# Autodesk Inventor assembly: KB33-046-004 - Внешний корпус
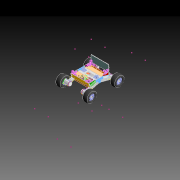
[picture p0: Inventor's stored thumbnail of the model, 180x180]
Saved by Autodesk Inventor 2020 (Build 240168000, 168)
## iProperties
Created: 2021-06-25
Part Number: KB33-046-004 - Внешний корпус
Document SubType Name: Assembly
Designer: Петров Иван
Mass: 3036.48 g
Surface Area: 14093.4 cm^2
Volume: 2856.02 cm^3
Density: 1.06319 g/cm^3
Author: Петров Иван
## Documents named in this file (32)
- E:\IVAN\Ivan_desktop\Kvantorium\Projects\RoboPatrol\design\KB33-046-004 - Внешний корпус.iam
- E:\IVAN\Ivan_desktop\Kvantorium\Projects\RoboPatrol\design\KB33-046-004-001 - Центральная пластина.ipt
- E:\IVAN\Ivan_desktop\Kvantorium\Projects\RoboPatrol\design\KB33-046-004-002 - Передняя пластина.ipt
- E:\IVAN\Ivan_desktop\Kvantorium\Projects\RoboPatrol\design\KB33-046-001 - Ходовая часть.iam
- E:\IVAN\Ivan_desktop\Kvantorium\Projects\RoboPatrol\design\KB33-046-004-003 - Задняя пластина.ipt
- E:\IVAN\Ivan_desktop\Kvantorium\Projects\RoboPatrol\design\KB33-046-004-004 - Центральная верхняя пластина.ipt
- E:\IVAN\Ivan_desktop\Kvantorium\Projects\RoboPatrol\design\KB33-046-004-005 - Лицевая наклонная пластина.ipt
- E:\IVAN\Ivan_desktop\Kvantorium\Projects\RoboPatrol\design\KB33-046-004-006 - Задняя наклонная пластина.ipt
- E:\IVAN\Ivan_desktop\Kvantorium\Projects\RoboPatrol\design\KB33-046-004-007 - Центральная левая боковая пластина.ipt
- E:\IVAN\Ivan_desktop\Kvantorium\Projects\RoboPatrol\design\KB33-046-004-008 - Центральная правая боковая пластина.ipt
- E:\IVAN\Ivan_desktop\Kvantorium\Projects\RoboPatrol\design\KB33-046-004-009 - Передняя левая боковая пластина.ipt
- E:\IVAN\Ivan_desktop\Kvantorium\Projects\RoboPatrol\design\KB33-046-004-010 - Передняя правая боковая пластина.ipt
- E:\IVAN\Ivan_desktop\Kvantorium\Projects\RoboPatrol\design\KB33-046-004-011 - Задняя правая боковая пластина.ipt
- E:\IVAN\Ivan_desktop\Kvantorium\Projects\RoboPatrol\design\KB33-046-004-012 - Задняя левая боковая пластина.ipt
- E:\IVAN\Ivan_desktop\Kvantorium\Projects\RoboPatrol\design\KB33-046-004-013 - Уголок.ipt
- E:\IVAN\Ivan_desktop\Kvantorium\Projects\RoboPatrol\design\KB33-046-004-013 - Уголок зеркальный.ipt
- E:\IVAN\Ivan_desktop\Kvantorium\Projects\RoboPatrol\design\standart_components\JetsonNano\Jetson nano_fixed.iam
- E:\IVAN\Ivan_desktop\Kvantorium\Projects\RoboPatrol\design\KB33-046-004-014 - Лицевая вертикальня пластина.ipt
- E:\IVAN\Ivan_desktop\Kvantorium\Projects\RoboPatrol\design\KB33-046-004-015 - Задняя вертикальня пластина.ipt
- E:\IVAN\Ivan_desktop\Kvantorium\Projects\RoboPatrol\design\KB33-046-004-016 - Крышка.ipt
- E:\IVAN\Ivan_desktop\Kvantorium\Projects\RoboPatrol\design\KB33-046-004-017 - Крышка наклонная.ipt
- E:\IVAN\Ivan_desktop\Kvantorium\Projects\RoboPatrol\design\KB33-046-004-018 - Полка электроники.ipt
- E:\IVAN\Ivan_desktop\Kvantorium\Projects\RoboPatrol\design\standart_components\Lidar\RPLIDAR A2.iam
- E:\IVAN\Ivan_desktop\Kvantorium\Projects\RoboPatrol\design\standart_components\L298N\L298N_V2.ipt
- E:\IVAN\Ivan_desktop\Kvantorium\Projects\RoboPatrol\design\KB33-046-004-019 - Площадка под драйверы.ipt
- E:\IVAN\Ivan_desktop\Kvantorium\Projects\RoboPatrol\design\KB33-046-005 - Контроллер СНУ.iam
- E:\IVAN\Ivan_desktop\Kvantorium\Projects\RoboPatrol\design\KB33-046-007 - Контроллер АКБ.iam
- E:\IVAN\Ivan_desktop\Kvantorium\Projects\RoboPatrol\design\standart_components\Realsense\D400\IntelRealsense_D435_Multibody.ipt
- E:\IVAN\Ivan_desktop\Kvantorium\Projects\RoboPatrol\design\KB33-046-004-020 - Крепление глубинной камеры.ipt
- E:\IVAN\Ivan_desktop\Kvantorium\Projects\RoboPatrol\design\standart_components\TP_LINK_MR3023.ipt
- E:\IVAN\Ivan_desktop\Kvantorium\Projects\RoboPatrol\design\KB33-046-009 - Колпак лидара.iam
- E:\IVAN\Ivan_desktop\Kvantorium\Projects\RoboPatrol\design\KB33-046-008 - Блок АКБ.iam
## Components (35 placed, 31 different names)
1. KB33-046-004-001 - Центральная пластина:1 — Совмещение:1, Совмещение:2, Совмещение:3
2. KB33-046-004-002 - Передняя пластина:1 — Совмещение:4, Совмещение:5, Совмещение:6, Совмещение:80, Совмещение:100
3. KB33-046-001 - Ходовая часть:1 [sub-assembly] — Совмещение:1, Совмещение:2, Совмещение:3, Совмещение:4, Совмещение:5, Совмещение:6, Совмещение:7, Совмещение:8, Совмещение:9, Совмещение:10, Совмещение:11, Совмещение:12, Заподлицо:1, Совмещение:13, Совмещение:15, Совмещение:16, Совмещение:18, Совмещение:19, Совмещение:20, Совмещение:21, Совмещение:22, Совмещение:23, Заподлицо:2, Совмещение:24, Совмещение:25, Совмещение:26, Совмещение:27, Совмещение:28, Совмещение:29, Совмещение:30, Совмещение:31, Совмещение:32, Совмещение:33, Совмещение:34, Касательность:2, Совмещение:61, Совмещение:62, Совмещение:72, Заподлицо:16, Совмещение:101, Совмещение:102, Совмещение:104, Совмещение:105
4. KB33-046-004-003 - Задняя пластина:1 — Совмещение:7, Совмещение:8, Совмещение:9, Совмещение:103
5. KB33-046-004-004 - Центральная верхняя пластина:1 — Совмещение:10, Совмещение:11, Совмещение:12, Совмещение:73
6. KB33-046-004-005 - Лицевая наклонная пластина:1 — Заподлицо:1, Совмещение:13, Совмещение:36, Совмещение:40, Совмещение:62, Совмещение:81
7. KB33-046-004-006 - Задняя наклонная пластина:1 — Совмещение:15, Совмещение:16, Совмещение:38, Совмещение:42, Совмещение:61
8. KB33-046-004-007 - Центральная левая боковая пластина:1 — Совмещение:18, Совмещение:19, Совмещение:20
9. KB33-046-004-008 - Центральная правая боковая пластина:1 — Совмещение:21, Совмещение:22, Совмещение:23, Заподлицо:11, Заподлицо:12, Заподлицо:14, Совмещение:54
10. KB33-046-004-009 - Передняя левая боковая пластина:1 — Заподлицо:2, Совмещение:33, Совмещение:34, Совмещение:35, Заподлицо:3
11. KB33-046-004-010 - Передняя правая боковая пластина:1 — Совмещение:24, Совмещение:25, Совмещение:26, Совмещение:39, Заподлицо:5
12. KB33-046-004-011 - Задняя правая боковая пластина:1 — Совмещение:27, Совмещение:28, Совмещение:29, Совмещение:37, Заподлицо:4
13. KB33-046-004-012 - Задняя левая боковая пластина:1 — Совмещение:30, Совмещение:31, Совмещение:32, Совмещение:41, Заподлицо:6
14. KB33-046-004-013 - Уголок:1 — Совмещение:35, Совмещение:36, Заподлицо:3, Угол:2
15. KB33-046-004-013 - Уголок:2 — Совмещение:37, Совмещение:38, Заподлицо:4, Совмещение:49, Совмещение:50, Заподлицо:15, Угол:4
16. KB33-046-004-013 - Уголок зеркальный:1 — Совмещение:39, Заподлицо:5, Совмещение:40, Заподлицо:8, Заподлицо:9, Совмещение:48, Совмещение:63, Совмещение:82
17. KB33-046-004-013 - Уголок зеркальный:2 — Совмещение:41, Заподлицо:6, Совмещение:42, Угол:1, Совмещение:64
18. Jetson nano_fixed:1 [sub-assembly] — Совмещение:55, Совмещение:92, Совмещение:93, Совмещение:95
19. KB33-046-004-014 - Лицевая вертикальня пластина:1 — Заподлицо:8, Заподлицо:9, Совмещение:48
20. KB33-046-004-015 - Задняя вертикальня пластина:1 — Совмещение:49, Совмещение:50, Заподлицо:10, Заподлицо:13
21. KB33-046-004-016 - Крышка:1 — Заподлицо:10, Заподлицо:12, Заподлицо:13, Совмещение:67, Касательность:3, Угол:3, Совмещение:98, Угол:6
22. KB33-046-004-017 - Крышка наклонная:1 — Заподлицо:11, Заподлицо:14, Совмещение:54
23. KB33-046-004-018 - Полка электроники:1 — Заподлицо:15, Совмещение:55, Совмещение:63, Совмещение:64, Совмещение:89, Совмещение:95, Заподлицо:21
24. RPLIDAR A2:1 [sub-assembly] — Совмещение:67, Касательность:3, Угол:3, Совмещение:99
25. L298N_V2:1 — Угол:4, Угол:5, Заподлицо:17, Совмещение:75, Совмещение:76, Совмещение:79
26. L298N_V2:2 — Угол:5, Заподлицо:18, Совмещение:74, Совмещение:76
27. KB33-046-004-019 - Площадка под драйверы:1 — Совмещение:72, Совмещение:73, Заподлицо:16, Заподлицо:17, Заподлицо:18, Совмещение:74, Совмещение:75, Совмещение:77, Совмещение:78
28. main_pcb.brd:1 [sub-assembly] — Совмещение:80, Совмещение:81, Совмещение:82, Совмещение:87, Заподлицо:19, Заподлицо:20
29. BATTERIES_CONTROLLER.brd:1 [sub-assembly] — Совмещение:87, Заподлицо:19, Заподлицо:20
30. IntelRealsense_D435_Multibody:1 — Совмещение:90, Совмещение:91
31. KB33-046-004-020 - Крепление глубинной камеры:1 — Совмещение:89, Совмещение:90, Совмещение:91, Совмещение:92, Совмещение:93, Заподлицо:21
32. TP_LINK_MR3023:1 — Совмещение:106, Совмещение:107, Угол:7
33. KB33-046-009 - Колпак лидара:1 [sub-assembly] — Совмещение:98, Совмещение:99, Угол:6, Совмещение:106, Совмещение:107, Угол:7
34. KB33-046-008 - Блок АКБ:1 [sub-assembly] — Совмещение:100, Совмещение:101, Совмещение:102
35. KB33-046-008 - Блок АКБ:2 [sub-assembly] — Совмещение:103, Совмещение:104, Совмещение:105
## Relationships (107: Mate 78, Flush 20, Angle 7, Tangent 2)
- Совмещение:1 [Mate]: KB33-046-004-001 - Центральная пластина:1 ↔ KB33-046-001 - Ходовая часть:1
- Совмещение:2 [Mate]: KB33-046-004-001 - Центральная пластина:1 ↔ KB33-046-001 - Ходовая часть:1
- Совмещение:3 [Mate]: KB33-046-004-001 - Центральная пластина:1 ↔ KB33-046-001 - Ходовая часть:1
- Совмещение:4 [Mate]: KB33-046-004-002 - Передняя пластина:1 ↔ KB33-046-001 - Ходовая часть:1
- Совмещение:5 [Mate]: KB33-046-004-002 - Передняя пластина:1 ↔ KB33-046-001 - Ходовая часть:1
- Совмещение:6 [Mate]: KB33-046-004-002 - Передняя пластина:1 ↔ KB33-046-001 - Ходовая часть:1
- Совмещение:7 [Mate]: KB33-046-001 - Ходовая часть:1 ↔ KB33-046-004-003 - Задняя пластина:1
- Совмещение:8 [Mate]: KB33-046-001 - Ходовая часть:1 ↔ KB33-046-004-003 - Задняя пластина:1
- Совмещение:9 [Mate]: KB33-046-001 - Ходовая часть:1 ↔ KB33-046-004-003 - Задняя пластина:1
- Совмещение:10 [Mate]: KB33-046-001 - Ходовая часть:1 ↔ KB33-046-004-004 - Центральная верхняя пластина:1
- Совмещение:11 [Mate]: KB33-046-001 - Ходовая часть:1 ↔ KB33-046-004-004 - Центральная верхняя пластина:1
- Совмещение:12 [Mate]: KB33-046-001 - Ходовая часть:1 ↔ KB33-046-004-004 - Центральная верхняя пластина:1
- Заподлицо:1 [Flush]: KB33-046-001 - Ходовая часть:1 ↔ KB33-046-004-005 - Лицевая наклонная пластина:1
- Совмещение:13 [Mate]: KB33-046-001 - Ходовая часть:1 ↔ KB33-046-004-005 - Лицевая наклонная пластина:1
- Совмещение:15 [Mate]: KB33-046-001 - Ходовая часть:1 ↔ KB33-046-004-006 - Задняя наклонная пластина:1
- Совмещение:16 [Mate]: KB33-046-001 - Ходовая часть:1 ↔ KB33-046-004-006 - Задняя наклонная пластина:1
- Совмещение:18 [Mate]: KB33-046-001 - Ходовая часть:1 ↔ KB33-046-004-007 - Центральная левая боковая пластина:1
- Совмещение:19 [Mate]: KB33-046-001 - Ходовая часть:1 ↔ KB33-046-004-007 - Центральная левая боковая пластина:1
- Совмещение:20 [Mate]: KB33-046-001 - Ходовая часть:1 ↔ KB33-046-004-007 - Центральная левая боковая пластина:1
- Совмещение:21 [Mate]: KB33-046-001 - Ходовая часть:1 ↔ KB33-046-004-008 - Центральная правая боковая пластина:1
- Совмещение:22 [Mate]: KB33-046-001 - Ходовая часть:1 ↔ KB33-046-004-008 - Центральная правая боковая пластина:1
- Совмещение:23 [Mate]: KB33-046-001 - Ходовая часть:1 ↔ KB33-046-004-008 - Центральная правая боковая пластина:1
- Заподлицо:2 [Flush]: KB33-046-001 - Ходовая часть:1 ↔ KB33-046-004-009 - Передняя левая боковая пластина:1
- Совмещение:24 [Mate]: KB33-046-001 - Ходовая часть:1 ↔ KB33-046-004-010 - Передняя правая боковая пластина:1
- Совмещение:25 [Mate]: KB33-046-001 - Ходовая часть:1 ↔ KB33-046-004-010 - Передняя правая боковая пластина:1
- Совмещение:26 [Mate]: KB33-046-001 - Ходовая часть:1 ↔ KB33-046-004-010 - Передняя правая боковая пластина:1
- Совмещение:27 [Mate]: KB33-046-001 - Ходовая часть:1 ↔ KB33-046-004-011 - Задняя правая боковая пластина:1
- Совмещение:28 [Mate]: KB33-046-001 - Ходовая часть:1 ↔ KB33-046-004-011 - Задняя правая боковая пластина:1
- Совмещение:29 [Mate]: KB33-046-001 - Ходовая часть:1 ↔ KB33-046-004-011 - Задняя правая боковая пластина:1
- Совмещение:30 [Mate]: KB33-046-001 - Ходовая часть:1 ↔ KB33-046-004-012 - Задняя левая боковая пластина:1
- Совмещение:31 [Mate]: KB33-046-001 - Ходовая часть:1 ↔ KB33-046-004-012 - Задняя левая боковая пластина:1
- Совмещение:32 [Mate]: KB33-046-001 - Ходовая часть:1 ↔ KB33-046-004-012 - Задняя левая боковая пластина:1
- Совмещение:33 [Mate]: KB33-046-001 - Ходовая часть:1 ↔ KB33-046-004-009 - Передняя левая боковая пластина:1
- Совмещение:34 [Mate]: KB33-046-001 - Ходовая часть:1 ↔ KB33-046-004-009 - Передняя левая боковая пластина:1
- Совмещение:35 [Mate]: KB33-046-004-009 - Передняя левая боковая пластина:1 ↔ KB33-046-004-013 - Уголок:1
- Совмещение:36 [Mate]: KB33-046-004-005 - Лицевая наклонная пластина:1 ↔ KB33-046-004-013 - Уголок:1
- Заподлицо:3 [Flush]: KB33-046-004-009 - Передняя левая боковая пластина:1 ↔ KB33-046-004-013 - Уголок:1
- Совмещение:37 [Mate]: KB33-046-004-011 - Задняя правая боковая пластина:1 ↔ KB33-046-004-013 - Уголок:2
- Совмещение:38 [Mate]: KB33-046-004-006 - Задняя наклонная пластина:1 ↔ KB33-046-004-013 - Уголок:2
- Заподлицо:4 [Flush]: KB33-046-004-011 - Задняя правая боковая пластина:1 ↔ KB33-046-004-013 - Уголок:2
- Совмещение:39 [Mate]: KB33-046-004-010 - Передняя правая боковая пластина:1 ↔ KB33-046-004-013 - Уголок зеркальный:1
- Заподлицо:5 [Flush]: KB33-046-004-010 - Передняя правая боковая пластина:1 ↔ KB33-046-004-013 - Уголок зеркальный:1
- Совмещение:40 [Mate]: KB33-046-004-005 - Лицевая наклонная пластина:1 ↔ KB33-046-004-013 - Уголок зеркальный:1
- Совмещение:41 [Mate]: KB33-046-004-012 - Задняя левая боковая пластина:1 ↔ KB33-046-004-013 - Уголок зеркальный:2
- Заподлицо:6 [Flush]: KB33-046-004-012 - Задняя левая боковая пластина:1 ↔ KB33-046-004-013 - Уголок зеркальный:2
- Совмещение:42 [Mate]: KB33-046-004-006 - Задняя наклонная пластина:1 ↔ KB33-046-004-013 - Уголок зеркальный:2
- Угол:1 [Angle] (0 deg): KB33-046-004-013 - Уголок зеркальный:2
- Угол:2 [Angle] (0 deg): KB33-046-004-013 - Уголок:1
- Касательность:2 [Tangent]: KB33-046-001 - Ходовая часть:1
- Заподлицо:8 [Flush]: KB33-046-004-013 - Уголок зеркальный:1 ↔ KB33-046-004-014 - Лицевая вертикальня пластина:1
- Заподлицо:9 [Flush]: KB33-046-004-013 - Уголок зеркальный:1 ↔ KB33-046-004-014 - Лицевая вертикальня пластина:1
- Совмещение:48 [Mate]: KB33-046-004-013 - Уголок зеркальный:1 ↔ KB33-046-004-014 - Лицевая вертикальня пластина:1
- Совмещение:49 [Mate]: KB33-046-004-013 - Уголок:2 ↔ KB33-046-004-015 - Задняя вертикальня пластина:1
- Совмещение:50 [Mate]: KB33-046-004-013 - Уголок:2 ↔ KB33-046-004-015 - Задняя вертикальня пластина:1
- Заподлицо:10 [Flush]: KB33-046-004-015 - Задняя вертикальня пластина:1 ↔ KB33-046-004-016 - Крышка:1
- Заподлицо:11 [Flush]: KB33-046-004-008 - Центральная правая боковая пластина:1 ↔ KB33-046-004-017 - Крышка наклонная:1
- Заподлицо:12 [Flush]: KB33-046-004-008 - Центральная правая боковая пластина:1 ↔ KB33-046-004-016 - Крышка:1
- Заподлицо:13 [Flush]: KB33-046-004-015 - Задняя вертикальня пластина:1 ↔ KB33-046-004-016 - Крышка:1
- Заподлицо:14 [Flush]: KB33-046-004-008 - Центральная правая боковая пластина:1 ↔ KB33-046-004-017 - Крышка наклонная:1
- Совмещение:54 [Mate]: KB33-046-004-008 - Центральная правая боковая пластина:1 ↔ KB33-046-004-017 - Крышка наклонная:1
- Заподлицо:15 [Flush]: KB33-046-004-013 - Уголок:2 ↔ KB33-046-004-018 - Полка электроники:1
- Совмещение:55 [Mate] (5 mm): Jetson nano_fixed:1 ↔ KB33-046-004-018 - Полка электроники:1
- Совмещение:61 [Mate]: KB33-046-001 - Ходовая часть:1 ↔ KB33-046-004-006 - Задняя наклонная пластина:1
- Совмещение:62 [Mate]: KB33-046-001 - Ходовая часть:1 ↔ KB33-046-004-005 - Лицевая наклонная пластина:1
- Совмещение:63 [Mate]: KB33-046-004-013 - Уголок зеркальный:1 ↔ KB33-046-004-018 - Полка электроники:1
- Совмещение:64 [Mate]: KB33-046-004-013 - Уголок зеркальный:2 ↔ KB33-046-004-018 - Полка электроники:1
- Совмещение:67 [Mate]: KB33-046-004-016 - Крышка:1 ↔ RPLIDAR A2:1
- Касательность:3 [Tangent]: KB33-046-004-016 - Крышка:1 ↔ RPLIDAR A2:1
- Угол:3 [Angle] (0 deg): KB33-046-004-016 - Крышка:1 ↔ RPLIDAR A2:1
- Угол:4 [Angle] (180 deg): KB33-046-004-013 - Уголок:2 ↔ L298N_V2:1
- Угол:5 [Angle] (180 deg): L298N_V2:1 ↔ L298N_V2:2
- Совмещение:72 [Mate] (4 mm): KB33-046-001 - Ходовая часть:1 ↔ KB33-046-004-019 - Площадка под драйверы:1
- Совмещение:73 [Mate]: KB33-046-004-004 - Центральная верхняя пластина:1 ↔ KB33-046-004-019 - Площадка под драйверы:1
- Заподлицо:16 [Flush]: KB33-046-001 - Ходовая часть:1 ↔ KB33-046-004-019 - Площадка под драйверы:1
- Заподлицо:17 [Flush]: L298N_V2:1 ↔ KB33-046-004-019 - Площадка под драйверы:1
- Заподлицо:18 [Flush]: L298N_V2:2 ↔ KB33-046-004-019 - Площадка под драйверы:1
- Совмещение:74 [Mate] (4 mm): L298N_V2:2 ↔ KB33-046-004-019 - Площадка под драйверы:1
- Совмещение:75 [Mate] (4 mm): L298N_V2:1 ↔ KB33-046-004-019 - Площадка под драйверы:1
- Совмещение:76 [Mate]: L298N_V2:1 ↔ L298N_V2:2
- Совмещение:77 [Mate]: KB33-046-004-019 - Площадка под драйверы:1
- Совмещение:78 [Mate]: KB33-046-004-019 - Площадка под драйверы:1
- Совмещение:79 [Mate]: L298N_V2:1
- Совмещение:80 [Mate] (5 mm): KB33-046-004-002 - Передняя пластина:1 ↔ main_pcb.brd:1
- Совмещение:81 [Mate] (10 mm): KB33-046-004-005 - Лицевая наклонная пластина:1 ↔ main_pcb.brd:1
- Совмещение:82 [Mate] (140 mm): KB33-046-004-013 - Уголок зеркальный:1 ↔ main_pcb.brd:1
- Совмещение:87 [Mate] (10 mm): main_pcb.brd:1 ↔ BATTERIES_CONTROLLER.brd:1
- Заподлицо:19 [Flush]: main_pcb.brd:1 ↔ BATTERIES_CONTROLLER.brd:1
- Заподлицо:20 [Flush]: main_pcb.brd:1 ↔ BATTERIES_CONTROLLER.brd:1
- Совмещение:89 [Mate]: KB33-046-004-018 - Полка электроники:1 ↔ KB33-046-004-020 - Крепление глубинной камеры:1
- Совмещение:90 [Mate]: IntelRealsense_D435_Multibody:1 ↔ KB33-046-004-020 - Крепление глубинной камеры:1
- Совмещение:91 [Mate]: IntelRealsense_D435_Multibody:1 ↔ KB33-046-004-020 - Крепление глубинной камеры:1
- Совмещение:92 [Mate] (5 mm): Jetson nano_fixed:1 ↔ KB33-046-004-020 - Крепление глубинной камеры:1
- Совмещение:93 [Mate]: Jetson nano_fixed:1 ↔ KB33-046-004-020 - Крепление глубинной камеры:1
- Совмещение:95 [Mate]: Jetson nano_fixed:1 ↔ KB33-046-004-018 - Полка электроники:1
- Заподлицо:21 [Flush]: KB33-046-004-018 - Полка электроники:1 ↔ KB33-046-004-020 - Крепление глубинной камеры:1
- Совмещение:98 [Mate]: KB33-046-004-016 - Крышка:1 ↔ KB33-046-009 - Колпак лидара:1
- Совмещение:99 [Mate]: RPLIDAR A2:1 ↔ KB33-046-009 - Колпак лидара:1
- Угол:6 [Angle] (0 deg): KB33-046-004-016 - Крышка:1 ↔ KB33-046-009 - Колпак лидара:1
- Совмещение:100 [Mate]: KB33-046-004-002 - Передняя пластина:1 ↔ KB33-046-008 - Блок АКБ:1
- Совмещение:101 [Mate]: KB33-046-001 - Ходовая часть:1 ↔ KB33-046-008 - Блок АКБ:1
- Совмещение:102 [Mate]: KB33-046-001 - Ходовая часть:1 ↔ KB33-046-008 - Блок АКБ:1
- Совмещение:103 [Mate]: KB33-046-004-003 - Задняя пластина:1 ↔ KB33-046-008 - Блок АКБ:2
- Совмещение:104 [Mate]: KB33-046-001 - Ходовая часть:1 ↔ KB33-046-008 - Блок АКБ:2
- Совмещение:105 [Mate]: KB33-046-001 - Ходовая часть:1 ↔ KB33-046-008 - Блок АКБ:2
- Совмещение:106 [Mate]: TP_LINK_MR3023:1 ↔ KB33-046-009 - Колпак лидара:1
- Совмещение:107 [Mate]: TP_LINK_MR3023:1 ↔ KB33-046-009 - Колпак лидара:1
- Угол:7 [Angle] (0 deg): TP_LINK_MR3023:1 ↔ KB33-046-009 - Колпак лидара:1
